# Autodesk Inventor assembly: Assembly1correct
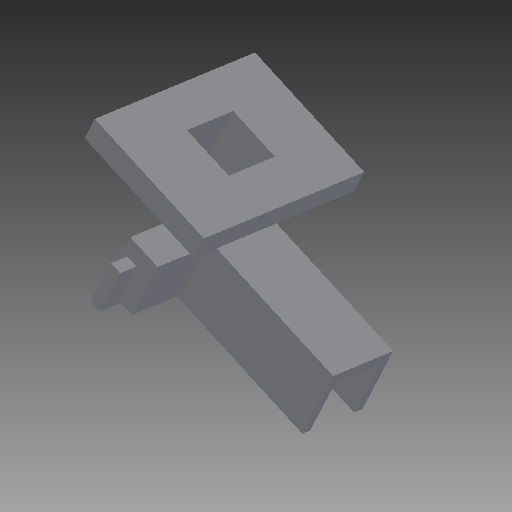
[picture p0: Inventor's stored thumbnail of the model, 512x512]
Saved by Autodesk Inventor 2019 (Build 230136000, 136)
## iProperties
Created: 2019-10-13
Part Number: Assembly1correct
Document SubType Name: Assembly
Designer: savan
Author: savan
## Documents named in this file (6)
- D:\my EE project subsystem\cup addition portion.iam
- D:\my EE project subsystem\addcup part 3 correct.ipt
- D:\my EE project subsystem\addcup part2 correct.ipt
- D:\my EE project subsystem\add cup base.ipt
- D:\my EE project subsystem\Part13.ipt
- D:\my EE project subsystem\Part12.ipt
## Components (5 placed, 5 different names)
1. addcup part 3 correct:1 — Rigid:2, Rigid:3, Rigid:4
2. addcup part2 correct:1 — Rigid:1, Rigid:2
3. add cup base:1 — Rigid:1
4. Part13:1 — Rigid:3
5. Part12:1 — Rigid:4
## Relationships (4: WeldJoint 4)
- Rigid:1 [WeldJoint]: addcup part2 correct:1 ↔ add cup base:1
- Rigid:2 [WeldJoint]: addcup part 3 correct:1 ↔ addcup part2 correct:1
- Rigid:3 [WeldJoint]: addcup part 3 correct:1 ↔ Part13:1
- Rigid:4 [WeldJoint]: addcup part 3 correct:1 ↔ Part12:1
